# Autodesk Inventor assembly: ASMCOMPLET
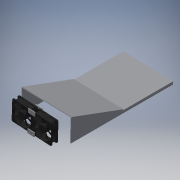
[picture p0: Inventor's stored thumbnail of the model, 180x180]
Saved by Autodesk Inventor 2017 (Build 210142000, 142)
## iProperties
Created: 2017-03-09
Part Number: ASMCOMPLET
Document SubType Name: Assembly
Designer: LaFaucheuse
Author: LaFaucheuse
## Documents named in this file (5)
- D:\[DATA]\[SW]\projetLDB\ASMCOMPLET.iam
- D:\[DATA]\[SW]\projetLDB\maquette.iam
- D:\[DATA]\[SW]\projetLDB\fanasm.iam
- D:\[DATA]\[SW]\projetLDB\cotelink.ipt
- D:\[DATA]\[SW]\projetLDB\top.ipt
## Components (5 placed, 4 different names)
1. maquette:1 [sub-assembly] — Placage:1, Placage:2, Placage:3, Placage:4, Placage:5, Placage:6
2. fanasm:1 [sub-assembly]
3. cotelink:1 — Placage:1, Placage:2, Placage:3, Placage:9, Placage:12
4. cotelink:2 — Placage:4, Placage:5, Placage:6, Placage:8, Placage:10, Placage:11
5. top:1 — Placage:8, Placage:9, Placage:10, Placage:11, Placage:12
## Relationships (11: Mate 11)
- Placage:1 [Mate]: maquette:1 ↔ cotelink:1
- Placage:2 [Mate]: maquette:1 ↔ cotelink:1
- Placage:3 [Mate]: maquette:1 ↔ cotelink:1
- Placage:4 [Mate]: maquette:1 ↔ cotelink:2
- Placage:5 [Mate]: maquette:1 ↔ cotelink:2
- Placage:6 [Mate]: maquette:1 ↔ cotelink:2
- Placage:8 [Mate]: cotelink:2 ↔ top:1
- Placage:9 [Mate]: cotelink:1 ↔ top:1
- Placage:10 [Mate]: cotelink:2 ↔ top:1
- Placage:11 [Mate]: cotelink:2 ↔ top:1
- Placage:12 [Mate]: cotelink:1 ↔ top:1
